# Autodesk Inventor assembly: A2017_T5_01
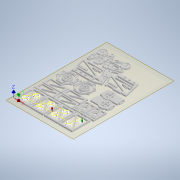
[picture p0: Inventor's stored thumbnail of the model, 180x180]
Saved by Autodesk Inventor 2020 (Build 240168000, 168)
## iProperties
Created: 2021-08-27
Part Number: A2017_T5_01
Document SubType Name: Assembly
Designer: Masato
Author: Masato
## Documents named in this file (12)
- C:\Users\naoki\Documents\Inventor\CitBrains\git_clone\OpenPlatform4_0\CAM\A2017_T5_01\OpenPlatform_ver3_0\cam\A2017_T5_01.iam
- C:\Users\naoki\Documents\Inventor\CitBrains\git_clone\OpenPlatform4_0\CAM\A2017_T5_01\OpenPlatform_ver3_0\cam\Disposable_Board.ipt
- C:\Users\naoki\Documents\Inventor\CitBrains\git_clone\OpenPlatform4_0\CAM\A2017_T5_01\OpenPlatform_ver3_0\LowerBody\Link\FrontLink_diagonal.ipt
- C:\Users\naoki\Documents\Inventor\CitBrains\git_clone\OpenPlatform4_0\CAM\A2017_T5_01\OpenPlatform_ver3_0\LowerBody\Link\BackLink_diagonal.ipt
- C:\Users\naoki\Documents\Inventor\CitBrains\git_clone\OpenPlatform4_0\CAM\A2017_T5_01\OpenPlatform_ver3_0\LowerBody\Knee\Knee_clamp.ipt
- C:\Users\naoki\Documents\Inventor\CitBrains\git_clone\OpenPlatform4_0\CAM\A2017_T5_01\OpenPlatform_ver3_0\LowerBody\Foot\Foot_root_block.ipt
- C:\Users\naoki\Documents\Inventor\CitBrains\git_clone\OpenPlatform4_0\CAM\A2017_T5_01\OpenPlatform_ver3_0\LowerBody\Ankle\Ankle_side_pitch_frame.ipt
- C:\Users\naoki\Documents\Inventor\CitBrains\git_clone\OpenPlatform4_0\CAM\A2017_T5_01\OpenPlatform_ver3_0\UpperBody\Arm\Shoulder_horn_frame.ipt
- C:\Users\naoki\Documents\Inventor\CitBrains\git_clone\OpenPlatform4_0\CAM\A2017_T5_01\OpenPlatform_ver3_0\UpperBody\Trunk\Trunk_lower_flank_frame.ipt
- C:\Users\naoki\Documents\Inventor\CitBrains\git_clone\OpenPlatform4_0\CAM\A2017_T5_01\OpenPlatform_ver3_0\LowerBody\Leg_joit\Leg_joint_yaw_frame.ipt
- C:\Users\naoki\Documents\Inventor\CitBrains\git_clone\OpenPlatform4_0\CAM\A2017_T5_01\OpenPlatform_ver3_0\UpperBody\Trunk\Inner_support_stand.ipt
- C:\Users\naoki\Documents\Inventor\CitBrains\git_clone\OpenPlatform4_0\CAM\A2017_T5_01\OpenPlatform_ver3_0\UpperBody\Trunk\Outer_support_stand.ipt
## Components (35 placed, 11 different names)
1. Disposable_Board:1 — メイト:2, メイト:1, フラッシュ:1, フラッシュ:2, フラッシュ:10, フラッシュ:11, 正接:13, フラッシュ:15, 角度:2, 角度:3
2. Ankle_side_pitch_frame:1 — フラッシュ:6, フラッシュ:16, 正接:18, メイト:33
3. Ankle_side_pitch_frame:2 — フラッシュ:8, メイト:33, 正接:19, 正接:20, 正接:21
4. Trunk_lower_flank_frame:1 — メイト:10, 正接:7, メイト:18, メイト:29, メイト:30, メイト:31, メイト:32, 角度:1
5. Trunk_lower_flank_frame:2 — メイト:10, 正接:7, メイト:17, 正接:16, 正接:17, フラッシュ:15, メイト:25, メイト:26, メイト:27, メイト:28, フラッシュ:16, 正接:18, 正接:19, 正接:22
6. Foot_root_block:1 — フラッシュ:9, メイト:24, メイト:29, メイト:30
7. Leg_joint_yaw_frame:1 — メイト:14, 正接:14, フラッシュ:13, フラッシュ:14, 正接:15
8. Leg_joint_yaw_frame:2 — メイト:13, フラッシュ:14, 正接:15
9. Inner_support_stand:1 — メイト:12, 挿入:1, 角度:2
10. Inner_support_stand:2 — メイト:15, 挿入:2, 角度:3
11. Outer_support_stand:1 — 正接:10, 正接:11, 正接:12, メイト:16, 挿入:2, 正接:17
12. Outer_support_stand:2 — 正接:8, 正接:9, 正接:12, 正接:13, メイト:11, 挿入:1, 正接:16
13. Foot_root_block:2 — メイト:22, メイト:25, メイト:26
14. Foot_root_block:3 — メイト:19, メイト:23, メイト:31, メイト:32
15. Foot_root_block:4 — メイト:21, メイト:27, メイト:28
16. Ankle_side_pitch_frame:3 — メイト:34, 正接:21, メイト:36, 正接:22, 角度:1
17. Ankle_side_pitch_frame:4 — メイト:34, 正接:20, メイト:35
18. FrontLink_diagonal:1 — メイト:4, フラッシュ:3, フラッシュ:4, フラッシュ:5, フラッシュ:6, フラッシュ:7, フラッシュ:8, フラッシュ:9, フラッシュ:10, 正接:1, 正接:2, 正接:3, 正接:4, 正接:5, 正接:6, フラッシュ:11, メイト:5, フラッシュ:12
19. Knee_clamp:1 — フラッシュ:3, 正接:4, 正接:5, 正接:6
20. Knee_clamp:2 — フラッシュ:4, 正接:1, 正接:2, 正接:3
21. FrontLink_diagonal:2
22. Knee_clamp:3
23. Knee_clamp:4
24. FrontLink_diagonal:3
25. Knee_clamp:5
26. Knee_clamp:6
27. FrontLink_diagonal:4 — メイト:6
28. Knee_clamp:7
29. Knee_clamp:8
30. BackLink_diagonal:1 — フラッシュ:5, メイト:5, フラッシュ:12
31. BackLink_diagonal:2 — 正接:8, 正接:9
32. BackLink_diagonal:3 — メイト:7
33. BackLink_diagonal:4 — 正接:10, 正接:11
34. Shoulder_horn_frame:1 — フラッシュ:7, メイト:6, メイト:7, フラッシュ:13
35. Shoulder_horn_frame:2 — 正接:14
## Component patterns: (4 elements, first: FrontLink_diagonal:1 + Knee_clamp:1 + Knee_clamp:2), (4 elements, first: BackLink_diagonal:1), (2 elements, first: Shoulder_horn_frame:1)
## Relationships (75: Mate 32, Tangent 22, Flush 16, Angle 3, Insert 2)
- メイト:2 [Mate]: Disposable_Board:1
- メイト:1 [Mate]: Disposable_Board:1
- フラッシュ:1 [Flush]: Disposable_Board:1
- フラッシュ:2 [Flush]: Disposable_Board:1
- メイト:4 [Mate]: FrontLink_diagonal:1
- フラッシュ:3 [Flush]: FrontLink_diagonal:1 ↔ Knee_clamp:1
- フラッシュ:4 [Flush]: FrontLink_diagonal:1 ↔ Knee_clamp:2
- フラッシュ:5 [Flush]: FrontLink_diagonal:1 ↔ BackLink_diagonal:1
- フラッシュ:6 [Flush]: Ankle_side_pitch_frame:1 ↔ FrontLink_diagonal:1
- フラッシュ:7 [Flush]: FrontLink_diagonal:1 ↔ Shoulder_horn_frame:1
- フラッシュ:8 [Flush]: Ankle_side_pitch_frame:2 ↔ FrontLink_diagonal:1
- フラッシュ:9 [Flush]: Foot_root_block:1 ↔ FrontLink_diagonal:1
- フラッシュ:10 [Flush] (2 mm): Disposable_Board:1 ↔ FrontLink_diagonal:1
- 正接:1 [Tangent] (2.5 mm): FrontLink_diagonal:1 ↔ Knee_clamp:2
- 正接:2 [Tangent] (2.5 mm): FrontLink_diagonal:1 ↔ Knee_clamp:2
- 正接:3 [Tangent] (2.5 mm): FrontLink_diagonal:1 ↔ Knee_clamp:2
- 正接:4 [Tangent] (2.5 mm): FrontLink_diagonal:1 ↔ Knee_clamp:1
- 正接:5 [Tangent] (2.5 mm): FrontLink_diagonal:1 ↔ Knee_clamp:1
- 正接:6 [Tangent] (2.5 mm): FrontLink_diagonal:1 ↔ Knee_clamp:1
- フラッシュ:11 [Flush] (2 mm): Disposable_Board:1 ↔ FrontLink_diagonal:1
- メイト:5 [Mate] (2.5 mm): FrontLink_diagonal:1 ↔ BackLink_diagonal:1
- フラッシュ:12 [Flush]: FrontLink_diagonal:1 ↔ BackLink_diagonal:1
- メイト:6 [Mate] (2.5 mm): FrontLink_diagonal:4 ↔ Shoulder_horn_frame:1
- メイト:7 [Mate] (2.5 mm): BackLink_diagonal:3 ↔ Shoulder_horn_frame:1
- メイト:10 [Mate] (2.5 mm): Trunk_lower_flank_frame:1 ↔ Trunk_lower_flank_frame:2
- 正接:7 [Tangent] (2.5 mm): Trunk_lower_flank_frame:1 ↔ Trunk_lower_flank_frame:2
- 正接:8 [Tangent] (2.5 mm): Outer_support_stand:2 ↔ BackLink_diagonal:2
- 正接:9 [Tangent] (2.5 mm): Outer_support_stand:2 ↔ BackLink_diagonal:2
- 正接:10 [Tangent] (2.5 mm): Outer_support_stand:1 ↔ BackLink_diagonal:4
- 正接:11 [Tangent] (2.5 mm): Outer_support_stand:1 ↔ BackLink_diagonal:4
- 正接:12 [Tangent] (2.5 mm): Outer_support_stand:1 ↔ Outer_support_stand:2
- 正接:13 [Tangent] (2.5 mm): Disposable_Board:1 ↔ Outer_support_stand:2
- メイト:11 [Mate]: Outer_support_stand:2
- メイト:12 [Mate]: Inner_support_stand:1
- メイト:13 [Mate]: Leg_joint_yaw_frame:2
- メイト:14 [Mate]: Leg_joint_yaw_frame:1
- メイト:15 [Mate]: Inner_support_stand:2
- メイト:16 [Mate]: Outer_support_stand:1
- メイト:17 [Mate]: Trunk_lower_flank_frame:2
- メイト:18 [Mate]: Trunk_lower_flank_frame:1
- メイト:19 [Mate]: Foot_root_block:3
- 正接:14 [Tangent] (2.5 mm): Leg_joint_yaw_frame:1 ↔ Shoulder_horn_frame:2
- フラッシュ:13 [Flush]: Leg_joint_yaw_frame:1 ↔ Shoulder_horn_frame:1
- フラッシュ:14 [Flush]: Leg_joint_yaw_frame:1 ↔ Leg_joint_yaw_frame:2
- 正接:15 [Tangent] (2.5 mm): Leg_joint_yaw_frame:1 ↔ Leg_joint_yaw_frame:2
- 挿入:1 [Insert]: Inner_support_stand:1 ↔ Outer_support_stand:2
- 挿入:2 [Insert]: Inner_support_stand:2 ↔ Outer_support_stand:1
- 正接:16 [Tangent] (2.5 mm): Trunk_lower_flank_frame:2 ↔ Outer_support_stand:2
- 正接:17 [Tangent] (2.5 mm): Trunk_lower_flank_frame:2 ↔ Outer_support_stand:1
- フラッシュ:15 [Flush] (2.5 mm): Disposable_Board:1 ↔ Trunk_lower_flank_frame:2
- メイト:21 [Mate]: Foot_root_block:4
- メイト:22 [Mate]: Foot_root_block:2
- メイト:23 [Mate]: Foot_root_block:3
- メイト:24 [Mate]: Foot_root_block:1
- メイト:25 [Mate] (2.5 mm): Trunk_lower_flank_frame:2 ↔ Foot_root_block:2
- メイト:26 [Mate] (2.5 mm): Trunk_lower_flank_frame:2 ↔ Foot_root_block:2
- メイト:27 [Mate] (2.5 mm): Trunk_lower_flank_frame:2 ↔ Foot_root_block:4
- メイト:28 [Mate] (2.5 mm): Trunk_lower_flank_frame:2 ↔ Foot_root_block:4
- メイト:29 [Mate] (2.5 mm): Trunk_lower_flank_frame:1 ↔ Foot_root_block:1
- メイト:30 [Mate] (2.5 mm): Trunk_lower_flank_frame:1 ↔ Foot_root_block:1
- メイト:31 [Mate] (2.5 mm): Trunk_lower_flank_frame:1 ↔ Foot_root_block:3
- メイト:32 [Mate] (2.5 mm): Trunk_lower_flank_frame:1 ↔ Foot_root_block:3
- フラッシュ:16 [Flush]: Ankle_side_pitch_frame:1 ↔ Trunk_lower_flank_frame:2
- 正接:18 [Tangent] (2.5 mm): Ankle_side_pitch_frame:1 ↔ Trunk_lower_flank_frame:2
- メイト:33 [Mate] (2.5 mm): Ankle_side_pitch_frame:1 ↔ Ankle_side_pitch_frame:2
- 正接:19 [Tangent] (2.5 mm): Ankle_side_pitch_frame:2 ↔ Trunk_lower_flank_frame:2
- メイト:34 [Mate] (2.5 mm): Ankle_side_pitch_frame:3 ↔ Ankle_side_pitch_frame:4
- 正接:20 [Tangent] (2.5 mm): Ankle_side_pitch_frame:2 ↔ Ankle_side_pitch_frame:4
- 正接:21 [Tangent] (2.5 mm): Ankle_side_pitch_frame:2 ↔ Ankle_side_pitch_frame:3
- メイト:35 [Mate]: Ankle_side_pitch_frame:4
- メイト:36 [Mate]: Ankle_side_pitch_frame:3
- 正接:22 [Tangent] (2.5 mm): Trunk_lower_flank_frame:2 ↔ Ankle_side_pitch_frame:3
- 角度:1 [Angle] (0 deg): Trunk_lower_flank_frame:1 ↔ Ankle_side_pitch_frame:3
- 角度:2 [Angle] (0 deg): Disposable_Board:1 ↔ Inner_support_stand:1
- 角度:3 [Angle] (0 deg): Disposable_Board:1 ↔ Inner_support_stand:2
